# Autodesk Inventor assembly: Performance Shaft
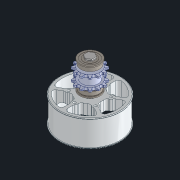
[picture p0: Inventor's stored thumbnail of the model, 180x180]
Saved by Autodesk Inventor 2022 (Build 260153000, 153)
## iProperties
Created: 2022-09-07
Part Number: Performance Shaft
Document SubType Name: Assembly
Designer: robpl
Author: robpl
## Documents named in this file (7)
- C:\Users\robpl\OneDrive\Documents\Inventor\2022 FRC Season\Best Coast Drive\Performance Shaft.iam
- C:\Users\robpl\OneDrive\Documents\Inventor\2022 FRC Season\Best Coast Drive\Performance Axle.ipt
- C:\Users\robpl\OneDrive\Documents\Inventor\2022 FRC Season\Best Coast Drive\0.5 Flanged Hex Bearing (1.125 OD) (217-3875).ipt
- C:\Users\robpl\OneDrive\Documents\Inventor\2022 FRC Season\Best Coast Drive\12T Steel Double Hub Sprocket (#35 Steel, 1_2_ Hex Bore) (217-5845) .ipt
- C:\Users\robpl\OneDrive\Documents\Inventor\2022 FRC Season\Best Coast Drive\am-4175 4IN Extrusion Performance Wheel 1.5IN Wide 500 hex.ipt
- C:\Users\robpl\OneDrive\Documents\Inventor\2022 FRC Season\Best Coast Drive\3mm 0.5in Hex Spacer.ipt
- C:\Users\robpl\OneDrive\Documents\Inventor\2022 FRC Season\Best Coast Drive\10mm E-Clip.ipt
## Components (10 placed, 6 different names)
1. Performance Axle:1 — Mate:1, Mate:2, Mate:3, Mate:4, Mate:5, Mate:6, Mate:8, Mate:9, Flush:1, Flush:2, Flush:3, Mate:15, Mate:17, Mate:18, Mate:19, Mate:20
2. 0.5 Flanged Hex Bearing (1.125 OD) (217-3875):1 — Mate:1, Mate:2, Flush:1, Mate:10, Mate:11, Mate:16
3. 0.5 Flanged Hex Bearing (1.125 OD) (217-3875):2 — Mate:5, Mate:6, Mate:13, Flush:2
4. 12T Steel Double Hub Sprocket (#35 Steel, 1_2_ Hex Bore) (217-5845) :1 — Mate:3, Mate:4, Mate:12, Mate:14
5. am-4175 4IN Extrusion Performance Wheel 1.5IN Wide 500 hex:1 — Mate:8, Mate:9, Flush:3
6. 3mm 0.5in Hex Spacer:1 — Mate:10, Mate:11, Mate:14
7. 3mm 0.5in Hex Spacer:2 — Mate:12, Mate:13
8. 10mm E-Clip:1 — Mate:15, Mate:16
9. 10mm E-Clip:2 — Mate:19, Mate:20
10. 10mm E-Clip:3 — Mate:17, Mate:18
## Relationships (22: Mate 19, Flush 3)
- Mate:1: Performance Axle:1 ↔ 0.5 Flanged Hex Bearing (1.125 OD) (217-3875):1
- Mate:2: Performance Axle:1 ↔ 0.5 Flanged Hex Bearing (1.125 OD) (217-3875):1
- Mate:3: Performance Axle:1 ↔ 12T Steel Double Hub Sprocket (#35 Steel, 1_2_ Hex Bore) (217-5845) :1
- Mate:4: Performance Axle:1 ↔ 12T Steel Double Hub Sprocket (#35 Steel, 1_2_ Hex Bore) (217-5845) :1
- Mate:5: Performance Axle:1 ↔ 0.5 Flanged Hex Bearing (1.125 OD) (217-3875):2
- Mate:6: Performance Axle:1 ↔ 0.5 Flanged Hex Bearing (1.125 OD) (217-3875):2
- Mate:8: Performance Axle:1 ↔ am-4175 4IN Extrusion Performance Wheel 1.5IN Wide 500 hex:1
- Mate:9: Performance Axle:1 ↔ am-4175 4IN Extrusion Performance Wheel 1.5IN Wide 500 hex:1
- Flush:1: Performance Axle:1 ↔ 0.5 Flanged Hex Bearing (1.125 OD) (217-3875):1
- Mate:10: 0.5 Flanged Hex Bearing (1.125 OD) (217-3875):1 ↔ 3mm 0.5in Hex Spacer:1
- Mate:11: 0.5 Flanged Hex Bearing (1.125 OD) (217-3875):1 ↔ 3mm 0.5in Hex Spacer:1
- Mate:12: 12T Steel Double Hub Sprocket (#35 Steel, 1_2_ Hex Bore) (217-5845) :1 ↔ 3mm 0.5in Hex Spacer:2
- Mate:13: 0.5 Flanged Hex Bearing (1.125 OD) (217-3875):2 ↔ 3mm 0.5in Hex Spacer:2
- Mate:14: 12T Steel Double Hub Sprocket (#35 Steel, 1_2_ Hex Bore) (217-5845) :1 ↔ 3mm 0.5in Hex Spacer:1
- Flush:2: Performance Axle:1 ↔ 0.5 Flanged Hex Bearing (1.125 OD) (217-3875):2
- Flush:3: Performance Axle:1 ↔ am-4175 4IN Extrusion Performance Wheel 1.5IN Wide 500 hex:1
- Mate:15: Performance Axle:1 ↔ 10mm E-Clip:1
- Mate:16: 0.5 Flanged Hex Bearing (1.125 OD) (217-3875):1 ↔ 10mm E-Clip:1
- Mate:17: Performance Axle:1 ↔ 10mm E-Clip:3
- Mate:18: Performance Axle:1 ↔ 10mm E-Clip:3
- Mate:19: Performance Axle:1 ↔ 10mm E-Clip:2
- Mate:20: Performance Axle:1 ↔ 10mm E-Clip:2
